# Autodesk Inventor assembly: 12v Pump
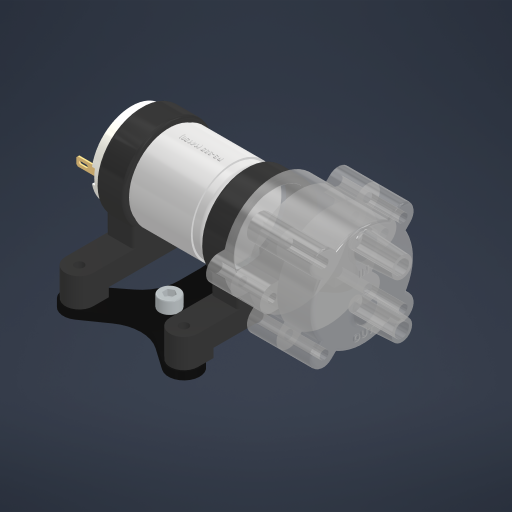
[picture p0: Inventor's stored thumbnail of the model, 512x512]
Saved by Autodesk Inventor 2024 (Build 280153000, 153)
## iProperties
Company: unknown
Created: 2018-07-10
Part Number: 12v Pump
Document SubType Name: Assembly
Designer: Vincent Larson
Sending System: unknown
Preprocessor: unknown
Minimum Resolution: 0.01
Sending System Product ID: 12V Diaphragm Pump v9
Sent Units: Millimeter
Translation Standard: IGES 5.3
Model Creation Time: 2018-07-10
Title: 12V Diaphragm Pump v9
Author: TekineticsLLC
## Documents named in this file (6)
- C:\Users\Vincent Larson\Downloads\12v Pump.iam
- C:\Users\Vincent Larson\Downloads\Motor_Main.ipt
- C:\Users\Vincent Larson\Downloads\Pump_Main.ipt
- C:\Users\Vincent Larson\Downloads\Rubber_Bracket.ipt
- C:\Users\Vincent Larson\Downloads\pump mount.ipt
- C:\Users\Vincent Larson\Downloads\Ender-3 Parts\01 MAIN ASM Ender_3\M4X10 Socket Head Screw.ipt
## Components (7 placed, 5 different names)
1. Motor_Main:1
2. Pump_Main:1
3. Rubber_Bracket:1 — Mate:2
4. Rubber_Bracket:2 — Mate:1
5. pump mount:1 — Mate:1, Mate:2, Mate:3, Mate:4, Mate:5
6. M4X10 Socket Head Screw:1 — Mate:3, Mate:5, Flush:1
7. M4X10 Socket Head Screw:2 — Mate:4, Flush:1
## Relationships (6: Mate 5, Flush 1)
- Mate:1: Rubber_Bracket:2 ↔ pump mount:1
- Mate:2: Rubber_Bracket:1 ↔ pump mount:1
- Mate:3: pump mount:1 ↔ M4X10 Socket Head Screw:1
- Mate:4: pump mount:1 ↔ M4X10 Socket Head Screw:2
- Mate:5: pump mount:1 ↔ M4X10 Socket Head Screw:1
- Flush:1: M4X10 Socket Head Screw:1 ↔ M4X10 Socket Head Screw:2
